# Autodesk Inventor assembly: F_Foot_v2
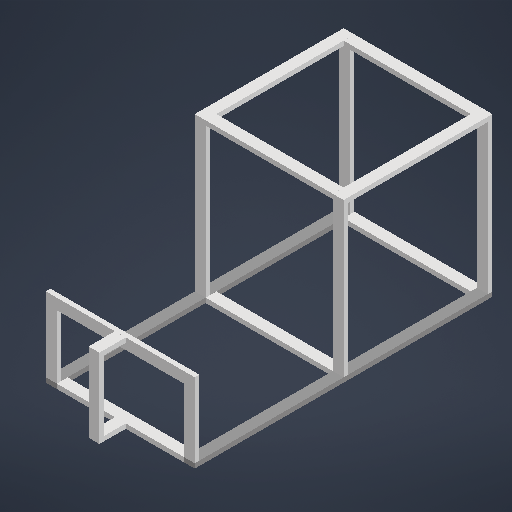
[picture p0: Inventor's stored thumbnail of the model, 512x512]
Saved by Autodesk Inventor 2027.1 (Build 311270010, 270A)
## iProperties
Created: 2026-08-30
Part Number: F_Foot_v2
Document SubType Name: Assembly
Designer: jorda
Author: jorda
## Documents named in this file (7)
- C:\Users\jorda\OneDrive\Documents\GitHub\USC-ASME-TigerBurn-2026\CAD\Legs\Front Foot\F_Foot_v2.iam
- C:\Users\jorda\OneDrive\Documents\GitHub\USC-ASME-TigerBurn-2026\CAD\Legs\Front Foot\2x4x48.ipt
- C:\Users\jorda\OneDrive\Documents\GitHub\USC-ASME-TigerBurn-2026\CAD\Legs\Front Foot\2x4x120.ipt
- C:\Users\jorda\OneDrive\Documents\GitHub\USC-ASME-TigerBurn-2026\CAD\Legs\Front Foot\2x4x41.ipt
- C:\Users\jorda\OneDrive\Documents\GitHub\USC-ASME-TigerBurn-2026\CAD\Legs\Front Foot\2x4x30.ipt
- C:\Users\jorda\OneDrive\Documents\GitHub\USC-ASME-TigerBurn-2026\CAD\Legs\Front Foot\2x4x8.5.ipt
- C:\Users\jorda\OneDrive\Documents\GitHub\USC-ASME-TigerBurn-2026\CAD\Legs\Front Foot\2x4x22.5.ipt
## Components (19 placed, 6 different names)
1. 2x4x120:1 — Mate:5, Flush:9, Flush:10, Mate:6, Flush:11, Flush:12, Flush:31, Mate:16, Flush:32, Flush:38, Flush:39
2. 2x4x48:2 — Mate:5, Flush:9, Flush:10, Mate:10, Flush:19, Flush:20
3. 2x4x120:2 — Mate:7, Flush:13, Flush:14, Mate:8, Flush:15, Flush:16, Mate:15, Flush:29, Mate:17, Flush:33, Flush:34, Flush:42
4. 2x4x48:3 — Mate:8, Flush:15, Flush:16, Mate:9, Flush:17, Flush:18
5. 2x4x41:1 — Mate:6, Flush:11, Flush:12
6. 2x4x41:2 — Mate:7, Flush:13, Flush:14, Flush:38, Flush:39, Flush:41, Mate:22
7. 2x4x48:4 — Mate:9, Flush:17, Flush:18, Mate:11, Flush:21, Flush:22, Mate:12, Flush:23, Flush:24, Mate:13, Flush:25, Flush:26
8. 2x4x48:5 — Mate:10, Flush:19, Flush:20, Mate:14, Flush:27, Flush:28
9. 2x4x41:3 — Mate:11, Flush:21, Flush:22
10. 2x4x41:4 — Mate:12, Flush:23, Flush:24
11. 2x4x48:6 — Mate:13, Flush:25, Flush:26, Flush:30
12. 2x4x48:7 — Mate:14, Flush:27, Flush:28
13. 2x4x41:5 — Mate:15, Flush:29, Flush:30
14. 2x4x30:1 — Flush:31, Mate:16, Flush:32, Mate:23
15. 2x4x30:2 — Mate:17, Flush:33, Flush:34, Flush:43
16. 2x4x8.5:1 — Flush:41, Mate:22, Flush:42, Flush:45
17. 2x4x41:7 — Flush:43, Mate:23, Flush:44, Mate:25
18. 2x4x8.5:2 — Flush:44, Mate:25, Flush:45, Mate:26, Flush:46, Flush:47
19. 2x4x22.5:1 — Mate:26, Flush:46, Flush:47
## Relationships (52: Flush 35, Mate 17)
- Mate:5: 2x4x120:1 ↔ 2x4x48:2
- Flush:9: 2x4x120:1 ↔ 2x4x48:2
- Flush:10: 2x4x120:1 ↔ 2x4x48:2
- Mate:6: 2x4x120:1 ↔ 2x4x41:1
- Flush:11: 2x4x120:1 ↔ 2x4x41:1
- Flush:12: 2x4x120:1 ↔ 2x4x41:1
- Mate:7: 2x4x120:2 ↔ 2x4x41:2
- Flush:13: 2x4x120:2 ↔ 2x4x41:2
- Flush:14: 2x4x120:2 ↔ 2x4x41:2
- Mate:8: 2x4x120:2 ↔ 2x4x48:3
- Flush:15: 2x4x120:2 ↔ 2x4x48:3
- Flush:16: 2x4x120:2 ↔ 2x4x48:3
- Mate:9: 2x4x48:3 ↔ 2x4x48:4
- Flush:17: 2x4x48:3 ↔ 2x4x48:4
- Flush:18: 2x4x48:3 ↔ 2x4x48:4
- Mate:10: 2x4x48:2 ↔ 2x4x48:5
- Flush:19: 2x4x48:2 ↔ 2x4x48:5
- Flush:20: 2x4x48:2 ↔ 2x4x48:5
- Mate:11: 2x4x48:4 ↔ 2x4x41:3
- Flush:21: 2x4x48:4 ↔ 2x4x41:3
- Flush:22: 2x4x48:4 ↔ 2x4x41:3
- Mate:12: 2x4x48:4 ↔ 2x4x41:4
- Flush:23: 2x4x48:4 ↔ 2x4x41:4
- Flush:24: 2x4x48:4 ↔ 2x4x41:4
- Mate:13: 2x4x48:4 ↔ 2x4x48:6
- Flush:25: 2x4x48:4 ↔ 2x4x48:6
- Flush:26: 2x4x48:4 ↔ 2x4x48:6
- Mate:14: 2x4x48:5 ↔ 2x4x48:7
- Flush:27: 2x4x48:5 ↔ 2x4x48:7
- Flush:28: 2x4x48:5 ↔ 2x4x48:7
- Mate:15: 2x4x120:2 ↔ 2x4x41:5
- Flush:29: 2x4x120:2 ↔ 2x4x41:5
- Flush:30: 2x4x48:6 ↔ 2x4x41:5
- Flush:31: 2x4x120:1 ↔ 2x4x30:1
- Mate:16: 2x4x120:1 ↔ 2x4x30:1
- Flush:32: 2x4x120:1 ↔ 2x4x30:1
- Mate:17: 2x4x120:2 ↔ 2x4x30:2
- Flush:33: 2x4x120:2 ↔ 2x4x30:2
- Flush:34: 2x4x120:2 ↔ 2x4x30:2
- Flush:38: 2x4x120:1 ↔ 2x4x41:2
- Flush:39: 2x4x120:1 ↔ 2x4x41:2
- Flush:41: 2x4x41:2 ↔ 2x4x8.5:1
- Mate:22: 2x4x41:2 ↔ 2x4x8.5:1
- Flush:42 (565.15 mm): 2x4x120:2 ↔ 2x4x8.5:1
- Flush:43: 2x4x30:2 ↔ 2x4x41:7
- Mate:23: 2x4x30:1 ↔ 2x4x41:7
- Flush:44: 2x4x41:7 ↔ 2x4x8.5:2
- Mate:25: 2x4x41:7 ↔ 2x4x8.5:2
- Flush:45: 2x4x8.5:1 ↔ 2x4x8.5:2
- Mate:26: 2x4x8.5:2 ↔ 2x4x22.5:1
- Flush:46: 2x4x8.5:2 ↔ 2x4x22.5:1
- Flush:47: 2x4x8.5:2 ↔ 2x4x22.5:1
